# Autodesk Inventor assembly: Antenna assy_90
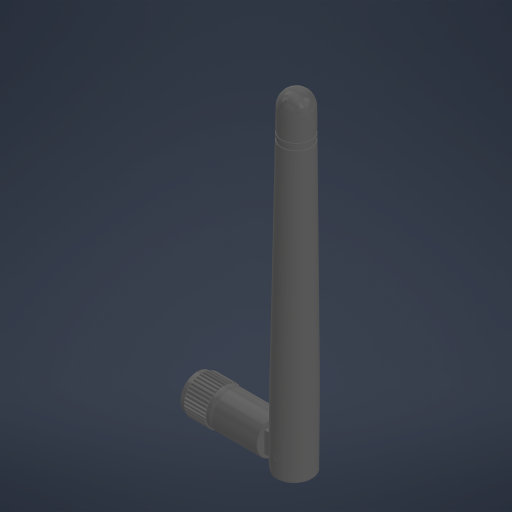
[picture p0: Inventor's stored thumbnail of the model, 512x512]
Saved by Autodesk Inventor 2024 (Build 280153000, 153)
## iProperties
Created: 2025-11-11
Part Number: Antenna assy_90
Document SubType Name: Assembly
Designer: Vincent Larson
Author: Vincent Larson
Revision Number: ANY
## Documents named in this file (3)
- C:\Users\Vincent Larson\Downloads\Digital Ship Challenge\Digital Ship Challenge Robot\NRF24L01L+Antenna\Antenna assy_90.iam
- C:\Users\Vincent Larson\Downloads\Digital Ship Challenge\Digital Ship Challenge Robot\NRF24L01L+Antenna\Antenna base.ipt
- C:\Users\Vincent Larson\Downloads\Digital Ship Challenge\Digital Ship Challenge Robot\NRF24L01L+Antenna\Antenna top.ipt
## Components (2 placed, 2 different names)
1. Antenna base_3 — Mate:1, Mate:2
2. Antenna top_4 — Mate:1, Mate:2
## Relationships (2: Mate 2)
- Mate:1: Antenna base_3 ↔ Antenna top_4
- Mate:2: Antenna base_3 ↔ Antenna top_4
